# Autodesk Inventor assembly: bumper
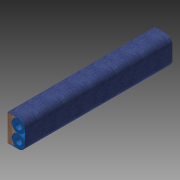
[picture p0: Inventor's stored thumbnail of the model, 180x180]
Saved by Autodesk Inventor 2015 SP1 (Build 190203100, 203)
## iProperties
Created: 2014-12-23
Part Number: bumper
Document SubType Name: Assembly
Designer: Jarod
Author: Jarod
## Documents named in this file (4)
- C:\Users\Jarod\Documents\Westview\Robotics\FRC\2015\CAD\Ideas\Square Frame\Square Frame Parts\bumper.iam
- C:\Users\Jarod\Documents\Westview\Robotics\FRC\2015\CAD\Ideas\Square Frame\Square Frame Parts\bumper_back.ipt
- C:\Users\Jarod\Documents\Westview\Robotics\FRC\2015\CAD\Ideas\Square Frame\Square Frame Parts\bumper_noodle.ipt
- C:\Users\Jarod\Documents\Westview\Robotics\FRC\2015\CAD\Ideas\Square Frame\Square Frame Parts\bumper_cloth.ipt
## Components (4 placed, 3 different names)
1. bumper_back:1 — Mate:1, Mate:2, Flush:1, Flush:2, Mate:3, Mate:4, Flush:3, Mate:5, Mate:6
2. bumper_noodle:1 — Mate:1, Mate:2, Flush:1
3. bumper_noodle:2 — Flush:2, Mate:3, Mate:4
4. bumper_cloth:1 — Flush:3, Mate:5, Mate:6
## Relationships (9: Mate 6, Flush 3)
- Mate:1 (31.75 mm): bumper_back:1 ↔ bumper_noodle:1
- Mate:2 (-31.75 mm): bumper_back:1 ↔ bumper_noodle:1
- Flush:1: bumper_back:1 ↔ bumper_noodle:1
- Flush:2: bumper_back:1 ↔ bumper_noodle:2
- Mate:3 (31.75 mm): bumper_back:1 ↔ bumper_noodle:2
- Mate:4 (-31.75 mm): bumper_back:1 ↔ bumper_noodle:2
- Flush:3: bumper_back:1 ↔ bumper_cloth:1
- Mate:5: bumper_back:1 ↔ bumper_cloth:1
- Mate:6: bumper_back:1 ↔ bumper_cloth:1
